# Autodesk Inventor assembly: Modul
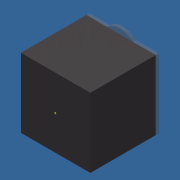
[picture p0: Inventor's stored thumbnail of the model, 180x180]
Saved by Autodesk Inventor 2018.2 (Build 222227000, 227)
## iProperties
Company: Fraunhofer ILT
Created: 2018-10-15
Part Number: Modul
Material: geeigneten Werkstoff auswählen !
Document SubType Name: Assembly
Designer: N.Grubert
Title: =Description
Author: N.Grubert
## Documents named in this file (3)
- C:\Users\GRUBERT\Documents\COSIMA-Laserstar\CAD\Modul.iam
- C:\Users\GRUBERT\Documents\COSIMA-Laserstar\CAD\Modul Deckel.ipt
- C:\Users\GRUBERT\Documents\COSIMA-Laserstar\CAD\Modul Gehäuse.ipt
## Components (2 placed, 2 different names)
1. Modul Deckel:1 — Passend:1, Fluchtend:1, Fluchtend:2
2. Modul Gehäuse:1 — Passend:1, Fluchtend:1, Fluchtend:2, Passend:2, Passend:3, Passend:4
## Relationships (6: Mate 4, Flush 2)
- Passend:1 [Mate]: Modul Deckel:1 ↔ Modul Gehäuse:1
- Fluchtend:1 [Flush]: Modul Deckel:1 ↔ Modul Gehäuse:1
- Fluchtend:2 [Flush]: Modul Deckel:1 ↔ Modul Gehäuse:1
- Passend:2 [Mate]: Modul Gehäuse:1
- Passend:3 [Mate]: Modul Gehäuse:1
- Passend:4 [Mate]: Modul Gehäuse:1
